# Autodesk Inventor assembly: Handle_2_rev2_Asm
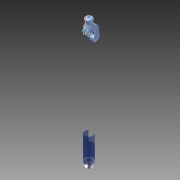
[picture p0: Inventor's stored thumbnail of the model, 180x180]
Saved by Autodesk Inventor 2011 SP2 (Build 150309200, 309)
## iProperties
Created: 2012-03-18
Part Number: Handle_2_rev2_Asm
Document SubType Name: Assembly
Designer: sungwook
Author: sungwook
## Documents named in this file (6)
- C:\Users\sungwook\Documents\Inventor\Micron20_Base_Tube_Adjst\Parts\Handle\Ver2(Al_RP)\Handle_2_rev2_Asm.iam
- C:\Users\sungwook\Documents\Inventor\Micron20_Base_Tube_Adjst\Parts\Handle\Ver2(Al_RP)\Main_Tubing_Al.ipt
- C:\Users\sungwook\Documents\Inventor\Micron20_Base_Tube_Adjst\Parts\Handle\Ver2(Al_RP)\Handle_2_Rev_Front.ipt
- C:\Users\sungwook\Documents\Inventor\Micron20\Parts\Handle\Ver2(Al_RP)\Handle_2_Back_Upper.ipt
- C:\Users\sungwook\Documents\Inventor\Micron20\Parts\Handle\Ver2(Al_RP)\Handle_2_Back_Bottom.ipt
- C:\Users\sungwook\Documents\Inventor\Micron20_Base_Tube_Adjst\Parts\Handle\Ver2(Al_RP)\Handle_2_Back_rev2.ipt
## Components (5 placed, 5 different names)
1. Main_Tubing_Al:1 — Flush:1, Mate:1, Mate:2, Flush:2, Flush:3, Mate:7, Mate:8, Mate:9, Mate:10
2. Handle_2_Rev_Front:1 — Flush:1, Mate:1, Mate:2
3. Handle_2_Back_Upper:1 — Flush:2, Mate:3, Mate:4, Mate:5, Mate:6, Mate:7, Mate:8
4. Handle_2_Back_Bottom:1 — Flush:3, Mate:3, Mate:4, Mate:5, Mate:6
5. Handle_2_Back_rev2:1 — Mate:9, Mate:10
## Relationships (13: Mate 10, Flush 3)
- Flush:1: Main_Tubing_Al:1 ↔ Handle_2_Rev_Front:1
- Mate:1: Main_Tubing_Al:1 ↔ Handle_2_Rev_Front:1
- Mate:2: Main_Tubing_Al:1 ↔ Handle_2_Rev_Front:1
- Flush:2: Main_Tubing_Al:1 ↔ Handle_2_Back_Upper:1
- Flush:3: Main_Tubing_Al:1 ↔ Handle_2_Back_Bottom:1
- Mate:3: Handle_2_Back_Upper:1 ↔ Handle_2_Back_Bottom:1
- Mate:4: Handle_2_Back_Upper:1 ↔ Handle_2_Back_Bottom:1
- Mate:5: Handle_2_Back_Upper:1 ↔ Handle_2_Back_Bottom:1
- Mate:6: Handle_2_Back_Upper:1 ↔ Handle_2_Back_Bottom:1
- Mate:7: Main_Tubing_Al:1 ↔ Handle_2_Back_Upper:1
- Mate:8: Main_Tubing_Al:1 ↔ Handle_2_Back_Upper:1
- Mate:9: Main_Tubing_Al:1 ↔ Handle_2_Back_rev2:1
- Mate:10: Main_Tubing_Al:1 ↔ Handle_2_Back_rev2:1
